# Autodesk Inventor assembly: Rail Stop
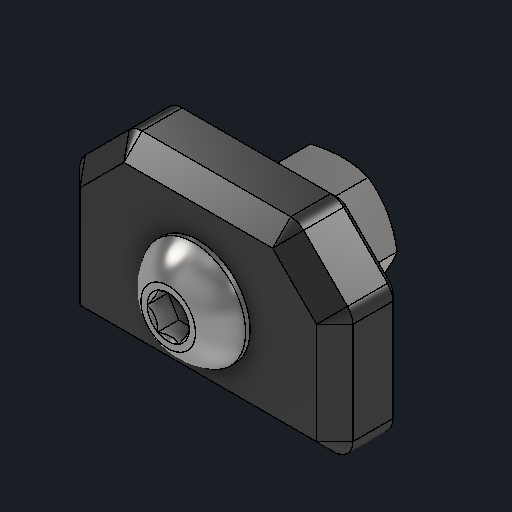
[picture p0: Inventor's stored thumbnail of the model, 512x512]
Saved by Autodesk Inventor 2026.1 (Build 301233020, 233B)
## iProperties
Created: 2025-05-11
Part Number: Rail Stop
Document SubType Name: Assembly
Designer: Joshua Eah
Author: Joshua Eah
## Documents named in this file (4)
- C:\Users\JoshuaEah\Documents\GitHub\Voron-0\CAD\Frame\Subassemblies\Rail Stop.iam
- C:\Users\JoshuaEah\Documents\GitHub\Voron-0\CAD\Hardware\M3x8 BHCS.ipt
- C:\Users\JoshuaEah\Documents\GitHub\Voron-0\CAD\Hardware\M3 Hexnut.ipt
- C:\Users\JoshuaEah\Documents\GitHub\Voron-0\CAD\Frame\Parts\Rail Stop.ipt
## Components (3 placed, 3 different names)
1. M3x8 BHCS:1 — Insert:1, Insert:2
2. M3 Hexnut:1 — Insert:2
3. Rail Stop:1 — Insert:1
## Relationships (2: Insert 2)
- Insert:1: M3x8 BHCS:1 ↔ Rail Stop:1
- Insert:2: M3x8 BHCS:1 ↔ M3 Hexnut:1
